# Autodesk Inventor assembly: tip2_ass_t1
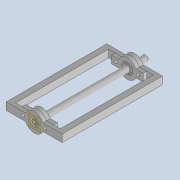
[picture p0: Inventor's stored thumbnail of the model, 180x180]
Saved by Autodesk Inventor 2020 (Build 240168000, 168)
## iProperties
Created: 2021-07-19
Part Number: tip2_ass_t1
Document SubType Name: Assembly
Designer: Shuang Peng
Author: Shuang Peng
## Documents named in this file (5)
- D:\projects-3\torque fb tip\hardware\tip_2\tip2_ass_t1.iam
- D:\projects-3\torque fb tip\hardware\tip_2\pin_3_60.ipt
- D:\projects-3\torque fb tip\hardware\tip_2\bearing_3_6_2.ipt
- D:\projects-3\torque fb tip\hardware\tip_2\cable_holder_1.ipt
- D:\projects-3\torque fb tip\hardware\tip_2\bearing_holder_2.ipt
## Components (6 placed, 4 different names)
1. pin_3_60:1 — Insert:7
2. cable_holder_1:1 — Flush:1, Insert:1, Insert:2, Insert:5, Insert:6, Insert:7
3. bearing_holder_2:1 — Flush:1, Insert:1, Insert:2, Insert:3
4. bearing_3_6_2:1 — Insert:3
5. bearing_holder_2:2 — Insert:5, Insert:6
6. bearing_3_6_2:2
## Relationships (8: Insert 7, Flush 1)
- Flush:1: cable_holder_1:1 ↔ bearing_holder_2:1
- Insert:1: cable_holder_1:1 ↔ bearing_holder_2:1
- Insert:2: cable_holder_1:1 ↔ bearing_holder_2:1
- Insert:3: bearing_holder_2:1 ↔ bearing_3_6_2:1
- [Insert]: bearing_holder_2:2 ↔ bearing_3_6_2:2
- Insert:5: cable_holder_1:1 ↔ bearing_holder_2:2
- Insert:6: cable_holder_1:1 ↔ bearing_holder_2:2
- Insert:7: pin_3_60:1 ↔ cable_holder_1:1
## Named parameters: d9_d8 = 0 mm
